# Autodesk Inventor assembly: Cube 1x1 V5 (USB Laser)
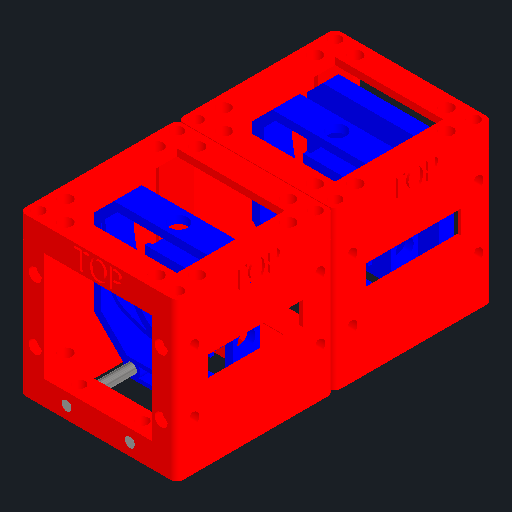
[picture p0: Inventor's stored thumbnail of the model, 512x512]
Saved by Autodesk Inventor 2023.4 (Build 274418000, 418)
## iProperties
Created: 2022-08-13
Part Number: Cube 1x1 V5 (USB Laser)
Document SubType Name: Assembly
Designer: xSibe
Author: xSibe
## Documents named in this file (5)
- C:\.Laptop\.Work\Projects\Project Protocube\Protocube\CAD, STL, OBJ Files\1 CAD\Laser\Cube 1x1 V5 (USB Laser).iam
- C:\.Laptop\.Work\Projects\Project Protocube\Protocube\CAD, STL, OBJ Files\1 CAD\Attachments\Mounting Bar.ipt
- C:\.Laptop\.Work\Projects\Project Protocube\Protocube\CAD, STL, OBJ Files\1 CAD\Filter\Filter Mount (SM1).ipt
- C:\.Laptop\.Work\Projects\Project Protocube\Protocube\CAD, STL, OBJ Files\1 CAD\Laser\Laser Holder (USB Laser).ipt
- C:\.Laptop\.Work\Projects\Project Protocube\Protocube\CAD, STL, OBJ Files\1 CAD\Cubes\Cube 1x1 V5 Laser.iam
## Components (7 placed, 4 different names)
1. Filter Mount (SM1):1 — Mate:4, Mate:5
2. Laser Holder (USB Laser):1
3. Mounting Bar:1 — Flush:1, Mate:4, Mate:5
4. Cube 1x1 V5 Laser:1 [sub-assembly]
5. Laser Holder (USB Laser):2
6. Mounting Bar:2
7. Cube 1x1 V5 Laser:2 [sub-assembly]
## Component patterns: (2 elements, first: Laser Holder (USB Laser):1 + Mounting Bar:1 + Cube 1x1 V5 Laser:1)
## Relationships (3: Mate 2, Flush 1)
- Flush:1: Mounting Bar:1
- Mate:4: Filter Mount (SM1):1 ↔ Mounting Bar:1
- Mate:5: Filter Mount (SM1):1 ↔ Mounting Bar:1
